# Autodesk Inventor assembly: inner_uper_glide_rod
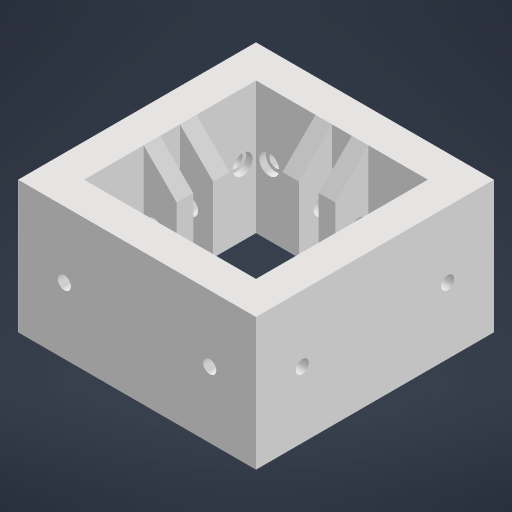
[picture p0: Inventor's stored thumbnail of the model, 512x512]
Saved by Autodesk Inventor 2024 (Build 280153000, 153)
## iProperties
Created: 2023-05-23
Part Number: inner_uper_glide_rod
Document SubType Name: Assembly
Designer: aasmu
Author: aasmu
## Documents named in this file (2)
- C:\Users\aasmu\Documents\standing_desk\inner_uper_glide_rod.iam
- C:\Users\aasmu\Documents\standing_desk\3_inner_glider_carriage_one_side.ipt
## Components (4 placed, 1 different names)
1. 3_inner_glider_carriage_one_side:1 — Rigid:2, Rigid:3
2. 3_inner_glider_carriage_one_side:2 — Rigid:3
3. 3_inner_glider_carriage_one_side:3 — Rigid:1
4. 3_inner_glider_carriage_one_side:4 — Rigid:1, Rigid:2
## Relationships (3: WeldJoint 3)
- Rigid:1 [WeldJoint]: 3_inner_glider_carriage_one_side:3 ↔ 3_inner_glider_carriage_one_side:4
- Rigid:2 [WeldJoint]: 3_inner_glider_carriage_one_side:1 ↔ 3_inner_glider_carriage_one_side:4
- Rigid:3 [WeldJoint]: 3_inner_glider_carriage_one_side:1 ↔ 3_inner_glider_carriage_one_side:2
